# Autodesk Inventor assembly: SHOULDER
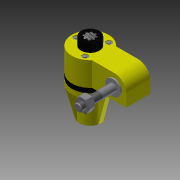
[picture p0: Inventor's stored thumbnail of the model, 180x180]
Saved by Autodesk Inventor 2013 (Build 170138000, 138)
## iProperties
Created: 2013-11-19
Part Number: SHOULDER
Document SubType Name: Assembly
Designer: employee
Author: employee
## Documents named in this file (9)
- C:\Users\employee\Desktop\ConceptFORGE\ConceptFORGE\LISA Simpson\INVENTOR FILES\SHOULDER.iam
- C:\Users\employee\Desktop\ConceptFORGE\ConceptFORGE\LISA Simpson\INVENTOR FILES\SHOULDER.ipt
- C:\Users\employee\Desktop\ConceptFORGE\ConceptFORGE\LISA Simpson\INVENTOR FILES\LEAD NUT.ipt
- C:\Users\employee\Desktop\ConceptFORGE\ConceptFORGE\LISA Simpson\INVENTOR FILES\M3 NUT.ipt
- C:\Users\employee\Desktop\ConceptFORGE\ConceptFORGE\LISA Simpson\INVENTOR FILES\M8x55.ipt
- C:\Users\employee\Desktop\ConceptFORGE\ConceptFORGE\LISA Simpson\INVENTOR FILES\M8 WASHER.ipt
- C:\Users\employee\Desktop\ConceptFORGE\ConceptFORGE\LISA Simpson\INVENTOR FILES\M8 NUT.ipt
- C:\Users\employee\Desktop\ConceptFORGE\ConceptFORGE\LISA Simpson\INVENTOR FILES\GUIDE.ipt
- C:\Users\employee\Desktop\ConceptFORGE\ConceptFORGE\LISA Simpson\INVENTOR FILES\M3x35.ipt
## Components (12 placed, 8 different names)
1. SHOULDER:1 — Insert:8, Angle:3, Insert:9, Insert:16, Mate:1, Insert:17, Insert:18, Insert:19, Angle:5, Angle:6, Angle:7, Mate:2
2. M3 NUT:1 — Insert:19, Angle:5
3. M3 NUT:2 — Insert:17, Angle:7
4. M3 NUT:3 — Insert:18, Angle:6
5. M8x55:1 — Insert:8, Angle:3
6. M8 WASHER:1 — Insert:9, Insert:10
7. M8 NUT:1 — Insert:10
8. GUIDE:1 — Insert:13, Insert:14, Insert:15, Insert:20
9. M3x35:1 — Insert:13, Mate:2
10. M3x35:2 — Insert:14
11. M3x35:3 — Insert:15
12. LEAD NUT:1 — Insert:16, Mate:1, Insert:20
## Relationships (17: Insert 11, Angle 4, Mate 2)
- Insert:8: SHOULDER:1 ↔ M8x55:1
- Angle:3 (0 deg): SHOULDER:1 ↔ M8x55:1
- Insert:9: SHOULDER:1 ↔ M8 WASHER:1
- Insert:10 (25 mm): M8 WASHER:1 ↔ M8 NUT:1
- Insert:13: GUIDE:1 ↔ M3x35:1
- Insert:14: GUIDE:1 ↔ M3x35:2
- Insert:15: GUIDE:1 ↔ M3x35:3
- Insert:16: SHOULDER:1 ↔ LEAD NUT:1
- Mate:1: SHOULDER:1 ↔ LEAD NUT:1
- Insert:17: SHOULDER:1 ↔ M3 NUT:2
- Insert:18: SHOULDER:1 ↔ M3 NUT:3
- Insert:19: SHOULDER:1 ↔ M3 NUT:1
- Angle:5 (0 deg): SHOULDER:1 ↔ M3 NUT:1
- Angle:6 (0 deg): SHOULDER:1 ↔ M3 NUT:3
- Angle:7 (0 deg): SHOULDER:1 ↔ M3 NUT:2
- Insert:20: GUIDE:1 ↔ LEAD NUT:1
- Mate:2: SHOULDER:1 ↔ M3x35:1
